# Autodesk Inventor assembly: disk
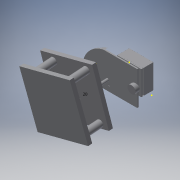
[picture p0: Inventor's stored thumbnail of the model, 180x180]
Saved by Autodesk Inventor 2019 (Build 230136000, 136)
## iProperties
Created: 2020-02-20
Part Number: disk
Document SubType Name: Assembly
Designer: ADMIN
Author: ADMIN
## Documents named in this file (9)
- C:\Users\Dell\Downloads\DISK THROWING MACHINE ASSEMBLED MODEL.iam
- C:\Users\Dell\Downloads\holder.ipt
- C:\Users\Dell\Downloads\glassplane.ipt
- C:\Users\Dell\Downloads\rod.ipt
- C:\Users\Dell\Downloads\wheel.ipt
- C:\Users\Dell\Downloads\base1.ipt
- C:\Users\Dell\Downloads\lowerbase.ipt
- C:\Users\Dell\Downloads\stepper.ipt
- C:\Users\Dell\Downloads\angle.ipt
## Components (8 placed, 8 different names)
1. holder:1
2. glassplane:1
3. rod:1 — Mate:1, Mate:2
4. wheel:1 — Mate:1
5. base1:1 — Mate:2
6. lowerbase:1
7. stepper:1
8. angle:1
## Relationships (2: Mate 2)
- Mate:1: rod:1 ↔ wheel:1
- Mate:2: rod:1 ↔ base1:1
